# Autodesk Inventor assembly: primary-engineer-bench
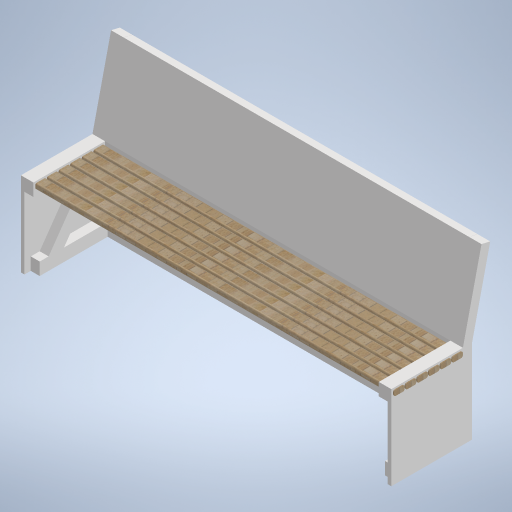
[picture p0: Inventor's stored thumbnail of the model, 512x512]
Saved by Autodesk Inventor 2023 (Build 270158030, 158C)
## iProperties
Created: 2024-09-09
Part Number: primary-engineer-bench
Document SubType Name: Assembly
Designer: Imogen Heard
Author: Imogen Heard
## Documents named in this file (6)
- C:\Users\dheard\Documents\0004-inventor\3D-CAD-main\primary-engineer-bench.iam
- C:\Users\dheard\Documents\0004-inventor\3D-CAD-main\bench-end-peice.ipt
- C:\Users\dheard\Documents\0004-inventor\3D-CAD-main\bench-slats.ipt
- C:\Users\dheard\Documents\0004-inventor\3D-CAD-main\bench-end-peice_MIR.ipt
- C:\Users\dheard\Documents\0004-inventor\3D-CAD-main\base-back.ipt
- C:\Users\dheard\Documents\0004-inventor\3D-CAD-main\backrest.ipt
## Components (5 placed, 5 different names)
1. bench-end-peice:1 — Flush:1, Symmetry:1, Flush:2, Flush:3, Flush:4, Flush:5
2. bench-slats:1 — Flush:1, Symmetry:1
3. bench-end-peice_MIR:1
4. base-back:1 — Flush:2, Flush:3
5. backrest:1 — Flush:4, Flush:5
## Relationships (6: Flush 5, Symmetry 1)
- Flush:1: bench-end-peice:1 ↔ bench-slats:1
- Symmetry:1: bench-end-peice:1 ↔ bench-slats:1
- Flush:2: bench-end-peice:1 ↔ base-back:1
- Flush:3: bench-end-peice:1 ↔ base-back:1
- Flush:4: bench-end-peice:1 ↔ backrest:1
- Flush:5: bench-end-peice:1 ↔ backrest:1
